# Autodesk Inventor assembly: ASSEMBLY
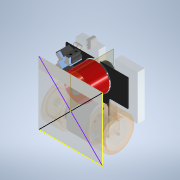
[picture p0: Inventor's stored thumbnail of the model, 180x180]
Saved by Autodesk Inventor 2020 (Build 240168000, 168)
## iProperties
Created: 2019-10-21
Part Number: ASSEMBLY
Document SubType Name: Assembly
Designer: atmat
Author: atmat
## Documents named in this file (18)
- D:\1.Projects\1.Roboty\2.JadeJager\Czesci\Ver 2\ASSEMBLY.iam
- D:\1.Projects\1.Roboty\2.JadeJager\Czesci\Ver 2\MOTOR_DETAL.ipt
- D:\1.Projects\1.Roboty\2.JadeJager\Czesci\Ver 2\GEAR_BOTTOM.ipt
- D:\1.Projects\1.Roboty\2.JadeJager\Czesci\Ver 2\GEAR_TOP.ipt
- D:\1.Projects\1.Roboty\2.JadeJager\Czesci\RACESTAR.ipt
- D:\1.Projects\1.Roboty\2.JadeJager\Czesci\Ver 2\Platworma_10x10.ipt
- D:\1.Projects\1.Roboty\2.JadeJager\Czesci\BLADE.ipt
- D:\1.Projects\1.Roboty\2.JadeJager\Czesci\Ver 2\Bateria_14V8.ipt
- D:\1.Projects\1.Roboty\2.JadeJager\Czesci\Ver 2\Kolo.ipt
- D:\1.Projects\1.Roboty\2.JadeJager\Czesci\Ver 2\Opona.ipt
- D:\1.Projects\1.Roboty\2.JadeJager\Czesci\Ver 2\Sharp_Czujnik_Linia.ipt
- D:\1.Projects\1.Roboty\2.JadeJager\Czesci\Ver 2\pcb.ipt
- D:\1.Projects\1.Roboty\2.JadeJager\Czesci\Ver 2\Hiolder_25.ipt
- D:\1.Projects\1.Roboty\2.JadeJager\Czesci\Ver 2\UberV2.ipt
- D:\1.Projects\1.Roboty\2.JadeJager\Czesci\Ver 2\LineBig.ipt
- D:\1.Projects\1.Roboty\2.JadeJager\Czesci\Ver 2\TX60.ipt
- D:\1.Projects\1.Roboty\2.JadeJager\Czesci\Ver 2\TX60_MIR.ipt
- D:\1.Projects\1.Roboty\2.JadeJager\Czesci\Ver 2\RadiatorCut.ipt
## Components (30 placed, 17 different names)
1. MOTOR_DETAL:1 — Tangent:28, Flush:18, Mate:56, Mate:59, Flush:20, Mate:61, Mate:63
2. GEAR_BOTTOM:1 — Mate:61, Mate:62, Mate:63, Mate:68
3. MOTOR_DETAL:2 — Tangent:28, Flush:18, Mate:53, Mate:54, Mate:55, Flush:19, Mate:58, Mate:60
4. GEAR_BOTTOM:3 — Mate:54, Mate:57, Mate:58, Mate:64
5. GEAR_TOP:2 — Flush:13, Mate:64, Mate:65, Flush:21
6. RACESTAR:1 — Mate:7, Mate:25, Mate:43, Mate:53, Mate:75
7. Platworma_10x10:1 — Mate:5, Flush:2, Mate:6, Mate:7, Mate:16, Mate:17, Flush:12, Flush:13, Flush:14, Mate:25, Mate:69, Tangent:29, Mate:75
8. BLADE:2 — Mate:5, Flush:2, Mate:6
9. Bateria_14V8:1 — Flush:24, Flush:25, Flush:27, Flush:35
10. GEAR_TOP:3 — Flush:14, Insert:3, Mate:68
11. Kolo:1 — Mate:65, Flush:21, Mate:66, Mate:67
12. Kolo:2 — Insert:3, Insert:5
13. Opona:1 — Mate:66, Mate:67, Tangent:29
14. Opona:2 — Insert:5
15. Sharp_Czujnik_Linia:7 — Mate:89, Flush:32, Angle:1, Mate:94
16. Sharp_Czujnik_Linia:4 — Mate:87, Mate:91, Mate:92, Angle:1, Angle:2, Mate:94, Mate:95
17. Sharp_Czujnik_Linia:5 — Mate:88, Mate:96, Angle:3
18. pcb:1 — Mate:43, Flush:22, Mate:81, Mate:82, Mate:83, Mate:84, Flush:23, Flush:24, Flush:25, Flush:26, Flush:28, Flush:31, Mate:87, Mate:88, Mate:89, Mate:90, Flush:32, Mate:91, Mate:92, Mate:93, Mate:97, Angle:4, Mate:98, Mate:99, Flush:33, Flush:34, Flush:35, Flush:36
19. Hiolder_25:1 — Mate:55, Mate:56, Flush:19, Mate:57, Mate:69, Mate:81
20. Hiolder_25:2 — Mate:59, Mate:60, Flush:20, Mate:62, Flush:22
21. UberV2:1 — Mate:84, Flush:29, Flush:30, Mate:85, Mate:86
22. UberV2:2 — Mate:83, Flush:30, Mate:86
23. UberV2:3 — Mate:82, Flush:28, Flush:29, Mate:85, Flush:31, Mate:100
24. Bateria_14V8:2 — Flush:23, Flush:26, Flush:27
25. Sharp_Czujnik_Linia:8 — Mate:90, Mate:93, Angle:2, Mate:95, Mate:96, Angle:3
26. LineBig:1 — Mate:97, Angle:4, Mate:98
27. LineBig:2
28. TX60:1 — Mate:99, Flush:33, Flush:34, Mate:101
29. TX60_MIR:1
30. RadiatorCut:1 — Mate:100, Flush:36, Mate:101
## Relationships (77: Mate 46, Flush 23, Angle 4, Insert 2, Tangent 2)
- Mate:5: Platworma_10x10:1 ↔ BLADE:2
- Flush:2: Platworma_10x10:1 ↔ BLADE:2
- Mate:6 (-18 mm): Platworma_10x10:1 ↔ BLADE:2
- Mate:7 (-50 mm): RACESTAR:1 ↔ Platworma_10x10:1
- Mate:16 (-1 mm): Platworma_10x10:1
- Mate:17 (-50 mm): Platworma_10x10:1
- Flush:12 (-50 mm): Platworma_10x10:1
- Flush:13 (0.5 mm): GEAR_TOP:2 ↔ Platworma_10x10:1
- Flush:14 (0.5 mm): Platworma_10x10:1 ↔ GEAR_TOP:3
- Mate:25 (3 mm): RACESTAR:1 ↔ Platworma_10x10:1
- Insert:3: GEAR_TOP:3 ↔ Kolo:2
- Insert:5: Kolo:2 ↔ Opona:2
- Mate:43: RACESTAR:1 ↔ pcb:1
- Tangent:28: MOTOR_DETAL:1 ↔ MOTOR_DETAL:2
- Flush:18: MOTOR_DETAL:1 ↔ MOTOR_DETAL:2
- Mate:53 (-18.25 mm): MOTOR_DETAL:2 ↔ RACESTAR:1
- Mate:54: MOTOR_DETAL:2 ↔ GEAR_BOTTOM:3
- Mate:55: MOTOR_DETAL:2 ↔ Hiolder_25:1
- Mate:56: MOTOR_DETAL:1 ↔ Hiolder_25:1
- Flush:19: MOTOR_DETAL:2 ↔ Hiolder_25:1
- Mate:57: GEAR_BOTTOM:3 ↔ Hiolder_25:1
- Mate:58: MOTOR_DETAL:2 ↔ GEAR_BOTTOM:3
- Mate:59: MOTOR_DETAL:1 ↔ Hiolder_25:2
- Mate:60: MOTOR_DETAL:2 ↔ Hiolder_25:2
- Flush:20: MOTOR_DETAL:1 ↔ Hiolder_25:2
- Mate:61: MOTOR_DETAL:1 ↔ GEAR_BOTTOM:1
- Mate:62: GEAR_BOTTOM:1 ↔ Hiolder_25:2
- Mate:63: MOTOR_DETAL:1 ↔ GEAR_BOTTOM:1
- Mate:64: GEAR_BOTTOM:3 ↔ GEAR_TOP:2
- Mate:65: GEAR_TOP:2 ↔ Kolo:1
- Flush:21: GEAR_TOP:2 ↔ Kolo:1
- Mate:66: Kolo:1 ↔ Opona:1
- Mate:67: Kolo:1 ↔ Opona:1
- Mate:68: GEAR_BOTTOM:1 ↔ GEAR_TOP:3
- Mate:69 (11.3 mm): Platworma_10x10:1 ↔ Hiolder_25:1
- Tangent:29 (-52.5 mm): Platworma_10x10:1 ↔ Opona:1
- Mate:75 (-23 mm): RACESTAR:1 ↔ Platworma_10x10:1
- Flush:22: pcb:1 ↔ Hiolder_25:2
- Mate:81: pcb:1 ↔ Hiolder_25:1
- Mate:82 (2.4 mm): pcb:1 ↔ UberV2:3
- Mate:83 (2.4 mm): pcb:1 ↔ UberV2:2
- Mate:84 (2.4 mm): pcb:1 ↔ UberV2:1
- Flush:23: pcb:1 ↔ Bateria_14V8:2
- Flush:24: Bateria_14V8:1 ↔ pcb:1
- Flush:25: Bateria_14V8:1 ↔ pcb:1
- Flush:26: pcb:1 ↔ Bateria_14V8:2
- Flush:27: Bateria_14V8:1 ↔ Bateria_14V8:2
- Flush:28: pcb:1 ↔ UberV2:3
- Flush:29: UberV2:1 ↔ UberV2:3
- Flush:30: UberV2:1 ↔ UberV2:2
- Mate:85: UberV2:1 ↔ UberV2:3
- Mate:86: UberV2:1 ↔ UberV2:2
- Flush:31 (11.1 mm): pcb:1 ↔ UberV2:3
- Mate:87: Sharp_Czujnik_Linia:4 ↔ pcb:1
- Mate:88: Sharp_Czujnik_Linia:5 ↔ pcb:1
- Mate:89: Sharp_Czujnik_Linia:7 ↔ pcb:1
- Mate:90: pcb:1 ↔ Sharp_Czujnik_Linia:8
- Flush:32: Sharp_Czujnik_Linia:7 ↔ pcb:1
- Mate:91: Sharp_Czujnik_Linia:4 ↔ pcb:1
- Mate:92: Sharp_Czujnik_Linia:4 ↔ pcb:1
- Mate:93: pcb:1 ↔ Sharp_Czujnik_Linia:8
- Angle:1 (225 deg): Sharp_Czujnik_Linia:7 ↔ Sharp_Czujnik_Linia:4
- Angle:2 (90 deg): Sharp_Czujnik_Linia:4 ↔ Sharp_Czujnik_Linia:8
- Mate:94 (1 mm): Sharp_Czujnik_Linia:7 ↔ Sharp_Czujnik_Linia:4
- Mate:95 (1 mm): Sharp_Czujnik_Linia:4 ↔ Sharp_Czujnik_Linia:8
- Mate:96: Sharp_Czujnik_Linia:5 ↔ Sharp_Czujnik_Linia:8
- Angle:3 (-135 deg): Sharp_Czujnik_Linia:5 ↔ Sharp_Czujnik_Linia:8
- Mate:97 (3 mm): pcb:1 ↔ LineBig:1
- Angle:4 (135 deg): pcb:1 ↔ LineBig:1
- Mate:98: pcb:1 ↔ LineBig:1
- Mate:99: pcb:1 ↔ TX60:1
- Flush:33: pcb:1 ↔ TX60:1
- Flush:34: pcb:1 ↔ TX60:1
- Flush:35 (25.1 mm): Bateria_14V8:1 ↔ pcb:1
- Mate:100: UberV2:3 ↔ RadiatorCut:1
- Flush:36: pcb:1 ↔ RadiatorCut:1
- Mate:101: TX60:1 ↔ RadiatorCut:1
